# Autodesk Inventor assembly: Petrischalenhalterung
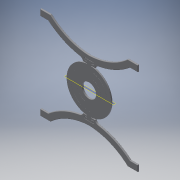
[picture p0: Inventor's stored thumbnail of the model, 180x180]
Saved by Autodesk Inventor 2018 (Build 220112000, 112)
## iProperties
Created: 2020-04-19
Part Number: Petrischalenhalterung
Material: Generisch
Document SubType Name: Assembly
Designer: maxse
Author: maxse
## Documents named in this file (6)
- C:\Users\maxse\Desktop\Bachelorarbeit\CAD-Dateien\Inventor Dateien\Petrischalenhalterung.iam
- C:\Users\maxse\Desktop\Bachelorarbeit\CAD-Dateien\Inventor Dateien\Fixierplatte_aussen_oben.ipt
- C:\Users\maxse\Desktop\Bachelorarbeit\CAD-Dateien\Inventor Dateien\Fixierplatte_aussen_unten.ipt
- C:\Users\maxse\Desktop\Bachelorarbeit\CAD-Dateien\Inventor Dateien\Fixierplatte_Innenring35mm.ipt
- C:\Users\maxse\Desktop\Bachelorarbeit\CAD-Dateien\Inventor Dateien\Fixierplatte_Innenring58,2mm.ipt
- C:\Users\maxse\Desktop\Bachelorarbeit\CAD-Dateien\Inventor Dateien\Fixierplatte_mitte.ipt
## Components (5 placed, 5 different names)
1. Fixierplatte_aussen_oben:1 — Passend:1, Passend:2, Winkel:1, Fluchtend:1
2. Fixierplatte_aussen_unten:1 — Passend:3, Passend:4, Fluchtend:2
3. Fixierplatte_Innenring35mm:1 — Passend:6, Passend:8
4. Fixierplatte_Innenring58,2mm:1 — Passend:5, Passend:6, Passend:7, Passend:8, Winkel:1, Fluchtend:1, Fluchtend:2
5. Fixierplatte_mitte:1 — Passend:1, Passend:2, Passend:3, Passend:4, Passend:5, Passend:7
## Relationships (11: Mate 8, Flush 2, Angle 1)
- Passend:1 [Mate]: Fixierplatte_aussen_oben:1 ↔ Fixierplatte_mitte:1
- Passend:2 [Mate]: Fixierplatte_aussen_oben:1 ↔ Fixierplatte_mitte:1
- Passend:3 [Mate]: Fixierplatte_aussen_unten:1 ↔ Fixierplatte_mitte:1
- Passend:4 [Mate]: Fixierplatte_aussen_unten:1 ↔ Fixierplatte_mitte:1
- Passend:5 [Mate]: Fixierplatte_Innenring58,2mm:1 ↔ Fixierplatte_mitte:1
- Passend:6 [Mate]: Fixierplatte_Innenring35mm:1 ↔ Fixierplatte_Innenring58,2mm:1
- Passend:7 [Mate]: Fixierplatte_Innenring58,2mm:1 ↔ Fixierplatte_mitte:1
- Passend:8 [Mate]: Fixierplatte_Innenring35mm:1 ↔ Fixierplatte_Innenring58,2mm:1
- Winkel:1 [Angle] (0 deg): Fixierplatte_aussen_oben:1 ↔ Fixierplatte_Innenring58,2mm:1
- Fluchtend:1 [Flush]: Fixierplatte_aussen_oben:1 ↔ Fixierplatte_Innenring58,2mm:1
- Fluchtend:2 [Flush]: Fixierplatte_aussen_unten:1 ↔ Fixierplatte_Innenring58,2mm:1
